# Autodesk Inventor assembly: Final Assembly
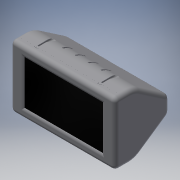
[picture p0: Inventor's stored thumbnail of the model, 180x180]
Saved by Autodesk Inventor 2018 (Build 220112000, 112)
## iProperties
Created: 2019-09-14
Part Number: Final Assembly
Document SubType Name: Assembly
Designer: Jacob
Author: Jacob
## Documents named in this file (3)
- C:\Users\Jacob\git_repos\POE-AIO\CAD Files\New Parts\Final Assembly.iam
- C:\Users\Jacob\git_repos\POE-AIO\CAD Files\New Parts\Display Assembly.iam
- C:\Users\Jacob\git_repos\POE-AIO\CAD Files\New Parts\Base Assembly.iam
## Components (2 placed, 2 different names)
1. Display Assembly:1 [sub-assembly]
2. Base Assembly:1 [sub-assembly]
## Relationships (3: Flush 2, Mate 1)
- [Mate]: Display Assembly:1 ↔ Base Assembly:1
- [Flush]: Display Assembly:1 ↔ Base Assembly:1
- [Flush]: Display Assembly:1 ↔ Base Assembly:1
